# Autodesk Inventor assembly: SM-GA01
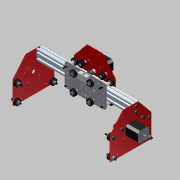
[picture p0: Inventor's stored thumbnail of the model, 180x180]
Saved by Autodesk Inventor 2012 SP1 (Build 160190100, 190)
## iProperties
Created: 2012-05-03
Part Number: SM-GA01
Document SubType Name: Assembly
Designer: ERF
Mass: 2383.97 g
Surface Area: 4504.24 cm^2
Volume: 551.69 cm^3
Density: 4.32122 g/cm^3
Author: ERF
Title: Shapeoko Gantry Assembly
Subject: Shapeoko Gantry Assembly
## Documents named in this file (7)
- C:\Users\eford\Documents\Projects\Shapoko_v1i\Workspaces\Workspace\Projects\USER FOLDER\Edward\Shapeoko_v1i\Assemblies\SM-GA01.iam
- C:\Users\eford\Documents\Projects\Shapoko_v1i\Workspaces\Workspace\Projects\USER FOLDER\Edward\Shapeoko_v1i\Parts\MSK01-02.ipt
- C:\Users\eford\Documents\Projects\Shapoko_v1i\Workspaces\Workspace\Projects\USER FOLDER\Edward\Shapeoko_v1i\Assemblies\SM-YA02.iam
- C:\Users\eford\Documents\Projects\Shapoko_v1i\Workspaces\Workspace\Projects\USER FOLDER\Edward\Shapeoko_v1i\Assemblies\SM-YA01.iam
- C:\Users\eford\Documents\Projects\Shapoko_v1i\Workspaces\Workspace\Projects\USER FOLDER\Edward\Shapeoko_v1i\Parts\SM-H07.ipt
- C:\Users\eford\Documents\Projects\Shapoko_v1i\Workspaces\Workspace\Projects\USER FOLDER\Edward\Shapeoko_v1i\Parts\SM-H03.ipt
- C:\Users\eford\Documents\Projects\Shapoko_v1i\Workspaces\Workspace\Projects\USER FOLDER\Edward\Shapeoko_v1i\Assemblies\SM-XZA1.iam
## Components (12 placed, 6 different names)
1. MSK01-02:1 — Insert:1, Insert:2, Insert:3, Insert:4, Mate:1, Flush:1
2. SM-YA02:1 [sub-assembly] — Insert:3, Insert:4, Insert:6, Insert:8
3. SM-YA01:1 [sub-assembly] — Insert:1, Insert:2, Insert:11, Insert:12
4. SM-H07:1 — Insert:9
5. SM-H07:2 — Insert:10
6. SM-H07:3 — Insert:5
7. SM-H07:4 — Insert:7
8. SM-H03:1 — Insert:10, Insert:11
9. SM-H03:2 — Insert:9, Insert:12
10. SM-H03:3 — Insert:5, Insert:6
11. SM-H03:4 — Insert:7, Insert:8
12. SM-XZA1:1 [sub-assembly] — Mate:1, Flush:1
## Relationships (14: Insert 12, Mate 1, Flush 1)
- Insert:1: MSK01-02:1 ↔ SM-YA01:1
- Insert:2: MSK01-02:1 ↔ SM-YA01:1
- Insert:3: MSK01-02:1 ↔ SM-YA02:1
- Insert:4: MSK01-02:1 ↔ SM-YA02:1
- Insert:5: SM-H07:3 ↔ SM-H03:3
- Insert:6: SM-YA02:1 ↔ SM-H03:3
- Insert:7: SM-H07:4 ↔ SM-H03:4
- Insert:8: SM-YA02:1 ↔ SM-H03:4
- Insert:9: SM-H07:1 ↔ SM-H03:2
- Insert:10: SM-H07:2 ↔ SM-H03:1
- Insert:11: SM-YA01:1 ↔ SM-H03:1
- Insert:12: SM-YA01:1 ↔ SM-H03:2
- Mate:1 (6.25 mm): MSK01-02:1 ↔ SM-XZA1:1
- Flush:1 (-25 mm): MSK01-02:1 ↔ SM-XZA1:1
